# Autodesk Inventor assembly: Carriage assy
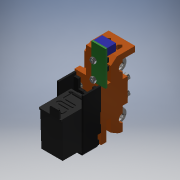
[picture p0: Inventor's stored thumbnail of the model, 180x180]
Saved by Autodesk Inventor 2018 (Build 220112000, 112)
## iProperties
Created: 2017-09-19
Part Number: Carriage assy
Document SubType Name: Assembly
Designer: Gabriel Smolnycki
Author: Gabriel Smolnycki
## Documents named in this file (13)
- H:\dev\planb\mechanics\V1INV\Subassemblies\Carriage assy.iam
- H:\dev\planb\mechanics\V1INV\Electronics\Cartridge Carrier.ipt
- H:\dev\planb\mechanics\V1INV\Electronics\C6602A.ipt
- H:\dev\planb\mechanics\V1INV\Carriage\Carriage Cartridge Adapter.ipt
- H:\dev\planb\mechanics\V1INV\Electronics\Endstop.ipt
- H:\dev\planb\mechanics\V1INV\Hardware\M3x10 SS SHCS.ipt
- H:\dev\planb\mechanics\V1INV\Hardware\M3 SS Nut.ipt
- H:\dev\planb\mechanics\V1INV\Carriage\Carriage Carrier.ipt
- H:\dev\planb\mechanics\V1INV\Hardware\8x25 Linear Bearing (63255K45).ipt
- H:\dev\planb\mechanics\V1INV\Carriage\Carriage Belt Clamp.ipt
- H:\dev\planb\mechanics\V1INV\Hardware\M4 SS Washer.ipt
- H:\dev\planb\mechanics\V1INV\Hardware\M4x30 SS SHCS.ipt
- H:\dev\planb\mechanics\V1INV\Hardware\M4 SS Locknut.ipt
## Components (25 placed, 12 different names)
1. Cartridge Carrier:1 — Insert:1, Insert:2, Mate:1, Mate:2, Tangent:1
2. C6602A:1 — Insert:1, Insert:2
3. Carriage Cartridge Adapter:1 — Insert:3, Insert:4, Insert:5, Insert:6, Insert:9, Insert:10, Mate:1, Mate:2, Tangent:1, Mate:5, Mate:6, Mate:7, Mate:8, Insert:23, Insert:24, Insert:25, Insert:26
4. Endstop:1 — Insert:3, Insert:4, Insert:7, Insert:8
5. M3x10 SS SHCS:1 — Insert:5
6. M3x10 SS SHCS:2 — Insert:6
7. M3 SS Nut:1 — Insert:7
8. M3 SS Nut:2 — Insert:8
9. Carriage Carrier:1 — Insert:9, Insert:10, Mate:3, Tangent:2, Mate:4, Tangent:3, Insert:11, Insert:12, Insert:13, Insert:14
10. 8x25 Linear Bearing (63255K45):1 — Mate:4, Tangent:3
11. 8x25 Linear Bearing (63255K45):2 — Mate:3, Tangent:2
12. Carriage Belt Clamp:1 — Insert:11, Insert:12, Insert:15, Insert:17
13. Carriage Belt Clamp:2 — Insert:13, Insert:14, Insert:16, Insert:18
14. M4 SS Washer:1 — Insert:16, Insert:21
15. M4 SS Washer:2 — Insert:17, Insert:20
16. M4 SS Washer:3 — Insert:18, Insert:22
17. M4 SS Washer:4 — Insert:15, Insert:19
18. M4x30 SS SHCS:1 — Insert:19
19. M4x30 SS SHCS:2 — Insert:20
20. M4x30 SS SHCS:3 — Insert:21
21. M4x30 SS SHCS:4 — Insert:22
22. M4 SS Locknut:1 — Mate:8, Insert:26
23. M4 SS Locknut:2 — Mate:7, Insert:24
24. M4 SS Locknut:3 — Mate:6, Insert:25
25. M4 SS Locknut:4 — Mate:5, Insert:23
## Relationships (37: Insert 26, Mate 8, Tangent 3)
- Insert:1: Cartridge Carrier:1 ↔ C6602A:1
- Insert:2: Cartridge Carrier:1 ↔ C6602A:1
- Insert:3: Carriage Cartridge Adapter:1 ↔ Endstop:1
- Insert:4: Carriage Cartridge Adapter:1 ↔ Endstop:1
- Insert:5: Carriage Cartridge Adapter:1 ↔ M3x10 SS SHCS:1
- Insert:6: Carriage Cartridge Adapter:1 ↔ M3x10 SS SHCS:2
- Insert:7: Endstop:1 ↔ M3 SS Nut:1
- Insert:8: Endstop:1 ↔ M3 SS Nut:2
- Insert:9: Carriage Cartridge Adapter:1 ↔ Carriage Carrier:1
- Insert:10: Carriage Cartridge Adapter:1 ↔ Carriage Carrier:1
- Mate:1: Cartridge Carrier:1 ↔ Carriage Cartridge Adapter:1
- Mate:2: Cartridge Carrier:1 ↔ Carriage Cartridge Adapter:1
- Tangent:1: Cartridge Carrier:1 ↔ Carriage Cartridge Adapter:1
- Mate:3: Carriage Carrier:1 ↔ 8x25 Linear Bearing (63255K45):2
- Tangent:2: Carriage Carrier:1 ↔ 8x25 Linear Bearing (63255K45):2
- Mate:4: Carriage Carrier:1 ↔ 8x25 Linear Bearing (63255K45):1
- Tangent:3: Carriage Carrier:1 ↔ 8x25 Linear Bearing (63255K45):1
- Insert:11: Carriage Carrier:1 ↔ Carriage Belt Clamp:1
- Insert:12: Carriage Carrier:1 ↔ Carriage Belt Clamp:1
- Insert:13: Carriage Carrier:1 ↔ Carriage Belt Clamp:2
- Insert:14: Carriage Carrier:1 ↔ Carriage Belt Clamp:2
- Insert:15: Carriage Belt Clamp:1 ↔ M4 SS Washer:4
- Insert:16: Carriage Belt Clamp:2 ↔ M4 SS Washer:1
- Insert:17: Carriage Belt Clamp:1 ↔ M4 SS Washer:2
- Insert:18: Carriage Belt Clamp:2 ↔ M4 SS Washer:3
- Insert:19: M4 SS Washer:4 ↔ M4x30 SS SHCS:1
- Insert:20: M4 SS Washer:2 ↔ M4x30 SS SHCS:2
- Insert:21: M4 SS Washer:1 ↔ M4x30 SS SHCS:3
- Insert:22: M4 SS Washer:3 ↔ M4x30 SS SHCS:4
- Mate:5: Carriage Cartridge Adapter:1 ↔ M4 SS Locknut:4
- Mate:6: Carriage Cartridge Adapter:1 ↔ M4 SS Locknut:3
- Mate:7: Carriage Cartridge Adapter:1 ↔ M4 SS Locknut:2
- Mate:8: Carriage Cartridge Adapter:1 ↔ M4 SS Locknut:1
- Insert:23: Carriage Cartridge Adapter:1 ↔ M4 SS Locknut:4
- Insert:24: Carriage Cartridge Adapter:1 ↔ M4 SS Locknut:2
- Insert:25: Carriage Cartridge Adapter:1 ↔ M4 SS Locknut:3
- Insert:26: Carriage Cartridge Adapter:1 ↔ M4 SS Locknut:1
